# Autodesk Inventor assembly: ASSY,INTAKE
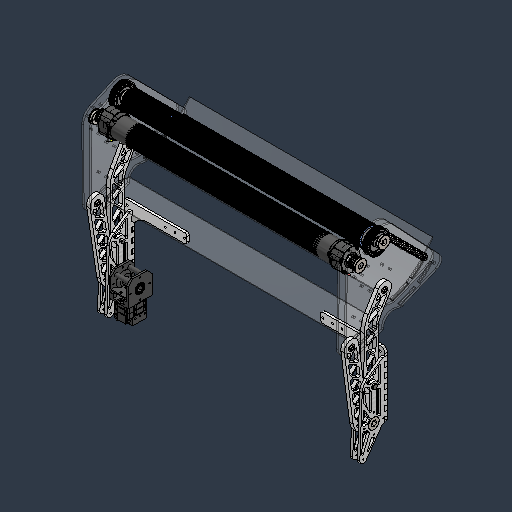
[picture p0: Inventor's stored thumbnail of the model, 512x512]
Saved by Autodesk Inventor 2026 (Build 300175050, 175E)
## iProperties
Created: 2026-02-09
Part Number: ASSY,INTAKE
Document SubType Name: Assembly
Designer: Jthib
Mass: 7601 g
Surface Area: 19123.7 cm^2
Volume: 4294.38 cm^3
Density: 1.76999 g/cm^3
Author: Jthib
## Documents named in this file (22)
- C:\Users\Jthib\Documents\GitHub\2026-Robot-Mechanical\Intake\ASSY,INTAKE.iam
- C:\Users\Jthib\Documents\GitHub\2026-Robot-Mechanical\Intake\PLATE,INTAKE,SIDE.ipt
- C:\Users\Jthib\Documents\GitHub\2026-Robot-Mechanical\#1_CAD Library\Power Transmission\Bearings\PURCHASED,HEX_BEARING.ipt
- C:\Users\Jthib\Documents\GitHub\2026-Robot-Mechanical\Intake\STOCK,HEX,INTAKE.ipt
- C:\Users\Jthib\Documents\GitHub\2026-Robot-Mechanical\Intake\PURCHASED,92320A546_18-8 Stainless Steel Unthreaded Spacer.ipt
- C:\Users\Jthib\Documents\GitHub\2026-Robot-Mechanical\#1_CAD Library\Electronics\CONTROLS,SPARK_FLEX.ipt
- C:\Users\Jthib\Documents\GitHub\2026-Robot-Mechanical\#1_CAD Library\Motors\MOTOR,REV,NEO,VORTEX.ipt
- C:\Users\Jthib\Documents\GitHub\2026-Robot-Mechanical\Intake\STOCK,CHURRO,LOWER,INTAKE.ipt
- C:\Users\Jthib\Documents\GitHub\2026-Robot-Mechanical\Intake\PLATE,HINGE,INTAKE,FRONT.ipt
- C:\Users\Jthib\Documents\GitHub\2026-Robot-Mechanical\Intake\PLATE,LINK,FRONT,INTAKE.ipt
- C:\Users\Jthib\Documents\GitHub\2026-Robot-Mechanical\Intake\PLATE,LINK,REAR,INTAKE.ipt
- C:\Users\Jthib\Documents\GitHub\2026-Robot-Mechanical\Intake\PURCHASED,20-1,90deg,MAX-PLANETARY.ipt
- C:\Users\Jthib\Documents\GitHub\2026-Robot-Mechanical\Intake\PURCHASED,6391K186_Oil-Embedded 841 Bronze Sleeve Bearing.ipt
- C:\Users\Jthib\Documents\GitHub\2026-Robot-Mechanical\Intake\PURCHASED,92390A271_18-8 Stainless Steel Clevis Pin.ipt
- C:\Users\Jthib\Documents\GitHub\2026-Robot-Mechanical\Intake\3DPRINT,SPACER,HEX,INTAKE.ipt
- C:\Users\Jthib\Documents\GitHub\2026-Robot-Mechanical\Intake\PURCHASED,2796T12_Ultra-Low-Friction Dry-Running Thrust Bearing.ipt
- C:\Users\Jthib\Documents\GitHub\2026-Robot-Mechanical\Intake\PLATE,CLAMP,MK4i,Swerve,CUSTOM,FRC2026.ipt
- C:\Users\Jthib\Documents\GitHub\2026-Robot-Mechanical\Intake\CAST,2inOD,ROLLER.ipt
- C:\Users\Jthib\Documents\GitHub\2026-Robot-Mechanical\#1_CAD Library\Power Transmission\Pulleys\PURCHASED,36T,HTD5mmx9mm,PULLEY.ipt
- C:\Users\Jthib\Documents\GitHub\2026-Robot-Mechanical\#1_CAD Library\Power Transmission\Pulleys\PURCHASED,15T,HTD5mmx9mm,PULLEY.ipt
- C:\Users\Jthib\Documents\GitHub\2026-Robot-Mechanical\Intake\PLATE,BOTTOM,BACK.ipt
- C:\Users\Jthib\Documents\GitHub\2026-Robot-Mechanical\Intake\PLATE,TOP,BACK.ipt
## Components (63 placed, 21 different names)
1. PLATE,INTAKE,SIDE:1 — Insert:20, Mate:46, Mate:48, Insert:26, Insert:28, Mate:50, Flush:53
2. PLATE,INTAKE,SIDE:2 — Insert:21, Mate:44, Mate:45, Insert:27, Insert:30, Mate:81
3. PLATE,INTAKE,SIDE:3 — Mate:31, Mate:32, Mate:33, Insert:24, Mate:51, Insert:31, Mate:86, Mate:90, Mate:92, Mate:93, Mate:94, Mate:95, Mate:96, Mate:97
4. PLATE,INTAKE,SIDE:4 — Insert:10, Mate:29, Mate:30, Mate:31, Mate:34, Insert:25, Insert:29, Flush:10
5. STOCK,HEX,INTAKE:1 — Mate:50, Flush:10, Mate:58, Mate:60, Mate:72, Mate:73, Mate:75, Mate:77, Mate:79
6. PURCHASED,92320A546_18-8 Stainless Steel Unthreaded Spacer:1 — Mate:43, Insert:20, Insert:21
7. PURCHASED,92320A546_18-8 Stainless Steel Unthreaded Spacer:2 — Mate:28, Mate:30, Mate:33, Mate:34
8. MOTOR,REV,NEO,VORTEX:1 — Insert:32, Mate:56
9. CONTROLS,SPARK_FLEX:1 — Mate:55, Insert:30, Insert:32, Mate:56
10. MOTOR,REV,NEO,VORTEX:2 — Mate:67
11. CONTROLS,SPARK_FLEX:2 — Mate:54, Insert:31
12. PURCHASED,HEX_BEARING:7 — Insert:26
13. PURCHASED,HEX_BEARING:8 — Insert:24, Mate:62
14. PURCHASED,HEX_BEARING:9 — Insert:25
15. PURCHASED,HEX_BEARING:10 — Insert:29
16. PURCHASED,92320A546_18-8 Stainless Steel Unthreaded Spacer:3 — Mate:42, Mate:44, Mate:45, Mate:46
17. PURCHASED,92320A546_18-8 Stainless Steel Unthreaded Spacer:4 — Mate:27, Insert:10, Mate:32
18. STOCK,CHURRO,LOWER,INTAKE:1 — Mate:95, Mate:96
19. PLATE,HINGE,INTAKE,FRONT:1 — Mate:19, Mate:20, Flush:1, Flush:2, Insert:1, Mate:24, Mate:26
20. PLATE,LINK,FRONT,INTAKE:1 — Insert:3, Flush:3, Insert:9
21. PLATE,LINK,REAR,INTAKE:1 — Mate:26, Flush:3, Insert:8, Mate:29
22. PURCHASED,6391K186_Oil-Embedded 841 Bronze Sleeve Bearing:1 — Insert:8, Mate:27
23. PURCHASED,92390A271_18-8 Stainless Steel Clevis Pin:1 — Insert:6
24. PLATE,HINGE,INTAKE,FRONT:2 — Mate:21, Mate:22, Flush:2, Insert:6, Mate:25, Insert:7
25. PURCHASED,6391K186_Oil-Embedded 841 Bronze Sleeve Bearing:2 — Insert:9, Mate:28
26. PURCHASED,HEX_BEARING:11 — Insert:7
27. PURCHASED,6391K186_Oil-Embedded 841 Bronze Sleeve Bearing:3 — Insert:3, Mate:24, Insert:4, Insert:5
28. 3DPRINT,SPACER,HEX,INTAKE:1 — Insert:1
29. PURCHASED,2796T12_Ultra-Low-Friction Dry-Running Thrust Bearing:1 — Insert:5
30. PURCHASED,2796T12_Ultra-Low-Friction Dry-Running Thrust Bearing:2 — Insert:4, Mate:25
31. PLATE,CLAMP,MK4i,Swerve,CUSTOM,FRC2026:1 — Mate:19, Mate:20, Flush:1, Mate:21, Mate:22, Flush:4, Flush:8, Mate:47
32. PLATE,CLAMP,MK4i,Swerve,CUSTOM,FRC2026:2 — Flush:4, Mate:35, Mate:36, Flush:5, Mate:37, Flush:6, Flush:8, Mate:47
33. PLATE,HINGE,INTAKE,FRONT:3 — Mate:37, Flush:6, Flush:7, Insert:16, Mate:40, Insert:17, Mate:41
34. PLATE,HINGE,INTAKE,FRONT:4 — Mate:35, Mate:36, Flush:5, Flush:7, Insert:11, Mate:39, Insert:15
35. PLATE,LINK,REAR,INTAKE:2 — Mate:40, Flush:9, Insert:18, Mate:48
36. PLATE,LINK,FRONT,INTAKE:2 — Insert:12, Flush:9, Insert:19
37. PURCHASED,6391K186_Oil-Embedded 841 Bronze Sleeve Bearing:4 — Insert:12, Insert:13, Insert:14, Mate:38
38. PURCHASED,6391K186_Oil-Embedded 841 Bronze Sleeve Bearing:5 — Insert:19, Mate:42
39. PURCHASED,6391K186_Oil-Embedded 841 Bronze Sleeve Bearing:6 — Insert:18, Mate:43
40. PURCHASED,2796T12_Ultra-Low-Friction Dry-Running Thrust Bearing:3 — Insert:14
41. PURCHASED,2796T12_Ultra-Low-Friction Dry-Running Thrust Bearing:4 — Insert:13, Mate:39
42. PURCHASED,92390A271_18-8 Stainless Steel Clevis Pin:2 — Insert:11, Mate:38
43. CAST,2inOD,ROLLER:1 — Mate:75, Mate:76, Mate:78
44. CAST,2inOD,ROLLER:2 — Mate:72, Mate:74, Mate:80
45. CAST,2inOD,ROLLER:3 — Mate:70, Mate:71
46. PURCHASED,20-1,90deg,MAX-PLANETARY:2 — Insert:17, Mate:41
47. PURCHASED,HEX_BEARING:12 — Insert:15
48. 3DPRINT,SPACER,HEX,INTAKE:2 — Insert:16
49. STOCK,HEX,INTAKE:2 — Mate:51, Flush:53, Mate:54, Mate:55, Mate:57, Mate:59, Mate:64, Mate:65, Mate:68, Mate:70
50. PURCHASED,36T,HTD5mmx9mm,PULLEY:1 — Mate:58, Flush:55, Mate:62
51. PURCHASED,36T,HTD5mmx9mm,PULLEY:2 — Mate:60, Mate:61, Flush:54
52. PURCHASED,15T,HTD5mmx9mm,PULLEY:1 — Mate:59, Flush:54
53. PURCHASED,15T,HTD5mmx9mm,PULLEY:2 — Mate:57, Flush:55
54. CAST,2inOD,ROLLER:4 — Mate:73, Mate:74, Mate:76
55. CAST,2inOD,ROLLER:6 — Mate:64, Mate:66, Mate:67
56. CAST,2inOD,ROLLER:7 — Mate:68, Mate:69, Mate:71
57. CAST,2inOD,ROLLER:8 — Mate:77, Mate:78, Mate:81
58. CAST,2inOD,ROLLER:9 — Mate:65, Mate:66, Mate:69
59. PLATE,BOTTOM,BACK:1 — Mate:90, Mate:92, Mate:97
60. PLATE,TOP,BACK:1 — Mate:86, Mate:93, Mate:94
61. PURCHASED,HEX_BEARING:13 — Insert:27, Mate:61
62. PURCHASED,HEX_BEARING:14 — Insert:28
63. CAST,2inOD,ROLLER:10 — Mate:79, Mate:80
## Relationships (111: Mate 69, Insert 29, Flush 13)
- [Mate]: MOTOR,REV,NEO,VORTEX:2 ↔ CONTROLS,SPARK_FLEX:2
- [Mate]: MOTOR,REV,NEO,VORTEX:2 ↔ CONTROLS,SPARK_FLEX:2
- [Mate]: MOTOR,REV,NEO,VORTEX:2 ↔ CONTROLS,SPARK_FLEX:2
- Mate:19: PLATE,HINGE,INTAKE,FRONT:1 ↔ PLATE,CLAMP,MK4i,Swerve,CUSTOM,FRC2026:1
- Mate:20 (0.1905 mm): PLATE,HINGE,INTAKE,FRONT:1 ↔ PLATE,CLAMP,MK4i,Swerve,CUSTOM,FRC2026:1
- Flush:1: PLATE,HINGE,INTAKE,FRONT:1 ↔ PLATE,CLAMP,MK4i,Swerve,CUSTOM,FRC2026:1
- Mate:21: PLATE,HINGE,INTAKE,FRONT:2 ↔ PLATE,CLAMP,MK4i,Swerve,CUSTOM,FRC2026:1
- Mate:22: PLATE,HINGE,INTAKE,FRONT:2 ↔ PLATE,CLAMP,MK4i,Swerve,CUSTOM,FRC2026:1
- Flush:2: PLATE,HINGE,INTAKE,FRONT:1 ↔ PLATE,HINGE,INTAKE,FRONT:2
- Insert:1: PLATE,HINGE,INTAKE,FRONT:1 ↔ 3DPRINT,SPACER,HEX,INTAKE:1
- Insert:3: PLATE,LINK,FRONT,INTAKE:1 ↔ PURCHASED,6391K186_Oil-Embedded 841 Bronze Sleeve Bearing:3
- Mate:24: PLATE,HINGE,INTAKE,FRONT:1 ↔ PURCHASED,6391K186_Oil-Embedded 841 Bronze Sleeve Bearing:3
- Insert:4: PURCHASED,6391K186_Oil-Embedded 841 Bronze Sleeve Bearing:3 ↔ PURCHASED,2796T12_Ultra-Low-Friction Dry-Running Thrust Bearing:2
- Insert:5: PURCHASED,6391K186_Oil-Embedded 841 Bronze Sleeve Bearing:3 ↔ PURCHASED,2796T12_Ultra-Low-Friction Dry-Running Thrust Bearing:1
- Insert:6: PURCHASED,92390A271_18-8 Stainless Steel Clevis Pin:1 ↔ PLATE,HINGE,INTAKE,FRONT:2
- Mate:25: PLATE,HINGE,INTAKE,FRONT:2 ↔ PURCHASED,2796T12_Ultra-Low-Friction Dry-Running Thrust Bearing:2
- Insert:7: PLATE,HINGE,INTAKE,FRONT:2 ↔ PURCHASED,HEX_BEARING:11
- Mate:26: PLATE,HINGE,INTAKE,FRONT:1 ↔ PLATE,LINK,REAR,INTAKE:1
- Flush:3: PLATE,LINK,FRONT,INTAKE:1 ↔ PLATE,LINK,REAR,INTAKE:1
- Insert:8: PLATE,LINK,REAR,INTAKE:1 ↔ PURCHASED,6391K186_Oil-Embedded 841 Bronze Sleeve Bearing:1
- Insert:9: PLATE,LINK,FRONT,INTAKE:1 ↔ PURCHASED,6391K186_Oil-Embedded 841 Bronze Sleeve Bearing:2
- Mate:27: PURCHASED,92320A546_18-8 Stainless Steel Unthreaded Spacer:4 ↔ PURCHASED,6391K186_Oil-Embedded 841 Bronze Sleeve Bearing:1
- Mate:28: PURCHASED,92320A546_18-8 Stainless Steel Unthreaded Spacer:2 ↔ PURCHASED,6391K186_Oil-Embedded 841 Bronze Sleeve Bearing:2
- Insert:10: PLATE,INTAKE,SIDE:4 ↔ PURCHASED,92320A546_18-8 Stainless Steel Unthreaded Spacer:4
- Mate:29 (3.175 mm): PLATE,INTAKE,SIDE:4 ↔ PLATE,LINK,REAR,INTAKE:1
- Mate:30: PLATE,INTAKE,SIDE:4 ↔ PURCHASED,92320A546_18-8 Stainless Steel Unthreaded Spacer:2
- Mate:31 (15.875 mm): PLATE,INTAKE,SIDE:3 ↔ PLATE,INTAKE,SIDE:4
- Mate:32: PLATE,INTAKE,SIDE:3 ↔ PURCHASED,92320A546_18-8 Stainless Steel Unthreaded Spacer:4
- Mate:33: PLATE,INTAKE,SIDE:3 ↔ PURCHASED,92320A546_18-8 Stainless Steel Unthreaded Spacer:2
- Mate:34: PLATE,INTAKE,SIDE:4 ↔ PURCHASED,92320A546_18-8 Stainless Steel Unthreaded Spacer:2
- Flush:4: PLATE,CLAMP,MK4i,Swerve,CUSTOM,FRC2026:1 ↔ PLATE,CLAMP,MK4i,Swerve,CUSTOM,FRC2026:2
- Mate:35: PLATE,CLAMP,MK4i,Swerve,CUSTOM,FRC2026:2 ↔ PLATE,HINGE,INTAKE,FRONT:4
- Mate:36 (0.1905 mm): PLATE,CLAMP,MK4i,Swerve,CUSTOM,FRC2026:2 ↔ PLATE,HINGE,INTAKE,FRONT:4
- Flush:5: PLATE,CLAMP,MK4i,Swerve,CUSTOM,FRC2026:2 ↔ PLATE,HINGE,INTAKE,FRONT:4
- Mate:37: PLATE,CLAMP,MK4i,Swerve,CUSTOM,FRC2026:2 ↔ PLATE,HINGE,INTAKE,FRONT:3
- Flush:6: PLATE,CLAMP,MK4i,Swerve,CUSTOM,FRC2026:2 ↔ PLATE,HINGE,INTAKE,FRONT:3
- Flush:7: PLATE,HINGE,INTAKE,FRONT:3 ↔ PLATE,HINGE,INTAKE,FRONT:4
- Flush:8: PLATE,CLAMP,MK4i,Swerve,CUSTOM,FRC2026:1 ↔ PLATE,CLAMP,MK4i,Swerve,CUSTOM,FRC2026:2
- Insert:11: PLATE,HINGE,INTAKE,FRONT:4 ↔ PURCHASED,92390A271_18-8 Stainless Steel Clevis Pin:2
- Insert:12: PLATE,LINK,FRONT,INTAKE:2 ↔ PURCHASED,6391K186_Oil-Embedded 841 Bronze Sleeve Bearing:4
- Insert:13: PURCHASED,6391K186_Oil-Embedded 841 Bronze Sleeve Bearing:4 ↔ PURCHASED,2796T12_Ultra-Low-Friction Dry-Running Thrust Bearing:4
- Insert:14: PURCHASED,6391K186_Oil-Embedded 841 Bronze Sleeve Bearing:4 ↔ PURCHASED,2796T12_Ultra-Low-Friction Dry-Running Thrust Bearing:3
- Mate:38: PURCHASED,6391K186_Oil-Embedded 841 Bronze Sleeve Bearing:4 ↔ PURCHASED,92390A271_18-8 Stainless Steel Clevis Pin:2
- Mate:39: PLATE,HINGE,INTAKE,FRONT:4 ↔ PURCHASED,2796T12_Ultra-Low-Friction Dry-Running Thrust Bearing:4
- Insert:15: PLATE,HINGE,INTAKE,FRONT:4 ↔ PURCHASED,HEX_BEARING:12
- Insert:16: PLATE,HINGE,INTAKE,FRONT:3 ↔ 3DPRINT,SPACER,HEX,INTAKE:2
- Mate:40: PLATE,HINGE,INTAKE,FRONT:3 ↔ PLATE,LINK,REAR,INTAKE:2
- Flush:9: PLATE,LINK,REAR,INTAKE:2 ↔ PLATE,LINK,FRONT,INTAKE:2
- Insert:17: PLATE,HINGE,INTAKE,FRONT:3 ↔ PURCHASED,20-1,90deg,MAX-PLANETARY:2
- Mate:41: PLATE,HINGE,INTAKE,FRONT:3 ↔ PURCHASED,20-1,90deg,MAX-PLANETARY:2
- Insert:18: PLATE,LINK,REAR,INTAKE:2 ↔ PURCHASED,6391K186_Oil-Embedded 841 Bronze Sleeve Bearing:6
- Insert:19: PLATE,LINK,FRONT,INTAKE:2 ↔ PURCHASED,6391K186_Oil-Embedded 841 Bronze Sleeve Bearing:5
- Mate:42: PURCHASED,92320A546_18-8 Stainless Steel Unthreaded Spacer:3 ↔ PURCHASED,6391K186_Oil-Embedded 841 Bronze Sleeve Bearing:5
- Mate:43: PURCHASED,92320A546_18-8 Stainless Steel Unthreaded Spacer:1 ↔ PURCHASED,6391K186_Oil-Embedded 841 Bronze Sleeve Bearing:6
- Insert:20: PLATE,INTAKE,SIDE:1 ↔ PURCHASED,92320A546_18-8 Stainless Steel Unthreaded Spacer:1
- Insert:21: PLATE,INTAKE,SIDE:2 ↔ PURCHASED,92320A546_18-8 Stainless Steel Unthreaded Spacer:1
- Mate:44: PLATE,INTAKE,SIDE:2 ↔ PURCHASED,92320A546_18-8 Stainless Steel Unthreaded Spacer:3
- Mate:45: PLATE,INTAKE,SIDE:2 ↔ PURCHASED,92320A546_18-8 Stainless Steel Unthreaded Spacer:3
- Mate:46: PLATE,INTAKE,SIDE:1 ↔ PURCHASED,92320A546_18-8 Stainless Steel Unthreaded Spacer:3
- Mate:47 (-698.5 mm): PLATE,CLAMP,MK4i,Swerve,CUSTOM,FRC2026:1 ↔ PLATE,CLAMP,MK4i,Swerve,CUSTOM,FRC2026:2
- Mate:48 (3.175 mm): PLATE,INTAKE,SIDE:1 ↔ PLATE,LINK,REAR,INTAKE:2
- Insert:24: PLATE,INTAKE,SIDE:3 ↔ PURCHASED,HEX_BEARING:8
- Insert:25: PLATE,INTAKE,SIDE:4 ↔ PURCHASED,HEX_BEARING:9
- Insert:26: PLATE,INTAKE,SIDE:1 ↔ PURCHASED,HEX_BEARING:7
- Insert:27: PLATE,INTAKE,SIDE:2 ↔ PURCHASED,HEX_BEARING:13
- Insert:28: PLATE,INTAKE,SIDE:1 ↔ PURCHASED,HEX_BEARING:14
- Mate:50: PLATE,INTAKE,SIDE:1 ↔ STOCK,HEX,INTAKE:1
- Insert:29: PLATE,INTAKE,SIDE:4 ↔ PURCHASED,HEX_BEARING:10
- Flush:10 (-0.127 mm): PLATE,INTAKE,SIDE:4 ↔ STOCK,HEX,INTAKE:1
- Mate:51: PLATE,INTAKE,SIDE:3 ↔ STOCK,HEX,INTAKE:2
- Flush:53 (-0.127 mm): PLATE,INTAKE,SIDE:1 ↔ STOCK,HEX,INTAKE:2
- Mate:54: CONTROLS,SPARK_FLEX:2 ↔ STOCK,HEX,INTAKE:2
- Mate:55: CONTROLS,SPARK_FLEX:1 ↔ STOCK,HEX,INTAKE:2
- Insert:30: PLATE,INTAKE,SIDE:2 ↔ CONTROLS,SPARK_FLEX:1
- Insert:31: PLATE,INTAKE,SIDE:3 ↔ CONTROLS,SPARK_FLEX:2
- Insert:32: MOTOR,REV,NEO,VORTEX:1 ↔ CONTROLS,SPARK_FLEX:1
- Mate:56: MOTOR,REV,NEO,VORTEX:1 ↔ CONTROLS,SPARK_FLEX:1
- Mate:57: STOCK,HEX,INTAKE:2 ↔ PURCHASED,15T,HTD5mmx9mm,PULLEY:2
- Mate:58: STOCK,HEX,INTAKE:1 ↔ PURCHASED,36T,HTD5mmx9mm,PULLEY:1
- Mate:59: STOCK,HEX,INTAKE:2 ↔ PURCHASED,15T,HTD5mmx9mm,PULLEY:1
- Mate:60: STOCK,HEX,INTAKE:1 ↔ PURCHASED,36T,HTD5mmx9mm,PULLEY:2
- Mate:61: PURCHASED,36T,HTD5mmx9mm,PULLEY:2 ↔ PURCHASED,HEX_BEARING:13
- Flush:54: PURCHASED,36T,HTD5mmx9mm,PULLEY:2 ↔ PURCHASED,15T,HTD5mmx9mm,PULLEY:1
- Flush:55: PURCHASED,36T,HTD5mmx9mm,PULLEY:1 ↔ PURCHASED,15T,HTD5mmx9mm,PULLEY:2
- Mate:62: PURCHASED,HEX_BEARING:8 ↔ PURCHASED,36T,HTD5mmx9mm,PULLEY:1
- Mate:64: STOCK,HEX,INTAKE:2 ↔ CAST,2inOD,ROLLER:6
- Mate:65: STOCK,HEX,INTAKE:2 ↔ CAST,2inOD,ROLLER:9
- Mate:66: CAST,2inOD,ROLLER:6 ↔ CAST,2inOD,ROLLER:9
- Mate:67 (-12.7 mm): MOTOR,REV,NEO,VORTEX:2 ↔ CAST,2inOD,ROLLER:6
- Mate:68: STOCK,HEX,INTAKE:2 ↔ CAST,2inOD,ROLLER:7
- Mate:69: CAST,2inOD,ROLLER:7 ↔ CAST,2inOD,ROLLER:9
- Mate:70: CAST,2inOD,ROLLER:3 ↔ STOCK,HEX,INTAKE:2
- Mate:71: CAST,2inOD,ROLLER:3 ↔ CAST,2inOD,ROLLER:7
- Mate:72: STOCK,HEX,INTAKE:1 ↔ CAST,2inOD,ROLLER:2
- Mate:73: STOCK,HEX,INTAKE:1 ↔ CAST,2inOD,ROLLER:4
- Mate:74: CAST,2inOD,ROLLER:2 ↔ CAST,2inOD,ROLLER:4
- Mate:75: STOCK,HEX,INTAKE:1 ↔ CAST,2inOD,ROLLER:1
- Mate:76: CAST,2inOD,ROLLER:1 ↔ CAST,2inOD,ROLLER:4
- Mate:77: STOCK,HEX,INTAKE:1 ↔ CAST,2inOD,ROLLER:8
- Mate:78: CAST,2inOD,ROLLER:1 ↔ CAST,2inOD,ROLLER:8
- Mate:79: STOCK,HEX,INTAKE:1 ↔ CAST,2inOD,ROLLER:10
- Mate:80: CAST,2inOD,ROLLER:2 ↔ CAST,2inOD,ROLLER:10
- Mate:81 (6.35 mm): PLATE,INTAKE,SIDE:2 ↔ CAST,2inOD,ROLLER:8
- Mate:86: PLATE,INTAKE,SIDE:3 ↔ PLATE,TOP,BACK:1
- Mate:90: PLATE,INTAKE,SIDE:3 ↔ PLATE,BOTTOM,BACK:1
- Mate:92: PLATE,INTAKE,SIDE:3 ↔ PLATE,BOTTOM,BACK:1
- Mate:93: PLATE,INTAKE,SIDE:3 ↔ PLATE,TOP,BACK:1
- Mate:94: PLATE,INTAKE,SIDE:3 ↔ PLATE,TOP,BACK:1
- Mate:95: PLATE,INTAKE,SIDE:3 ↔ STOCK,CHURRO,LOWER,INTAKE:1
- Mate:96: PLATE,INTAKE,SIDE:3 ↔ STOCK,CHURRO,LOWER,INTAKE:1
- Mate:97: PLATE,INTAKE,SIDE:3 ↔ PLATE,BOTTOM,BACK:1
## Named parameters: d94_d25 = 0 mm, d95_d26 = 0 mm, d96_d91_d27 = 0 mm
